# Autodesk Inventor assembly: vertical plate ass
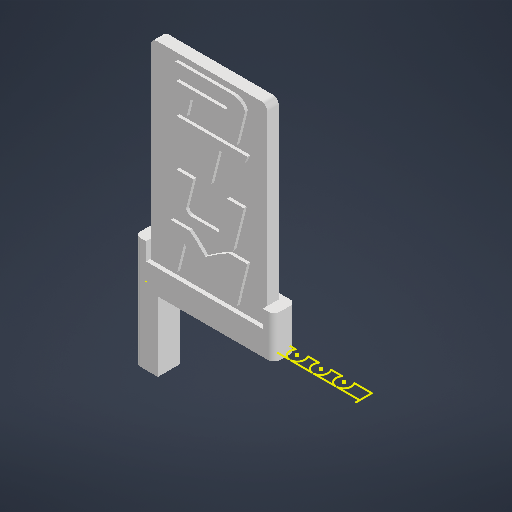
[picture p0: Inventor's stored thumbnail of the model, 512x512]
Saved by Autodesk Inventor 2025.1 (Build 291241000, 241)
## iProperties
Created: 2025-01-21
Part Number: vertical plate ass
Document SubType Name: Assembly
Designer: Juanl
Author: Juanl
## Documents named in this file (3)
- C:\Users\Juanl\Documents\GitHub\ATUM-V5RC-High-Stakes-CAD\Protobot\Hunter Mathis\vertical plate ass.iam
- C:\Users\Juanl\Documents\GitHub\ATUM-V5RC-High-Stakes-CAD\Protobot\Hunter Mathis\plate holder vertical.ipt
- C:\Users\Juanl\Documents\GitHub\ATUM-V5RC-High-Stakes-CAD\Protobot\Hunter Mathis\custom  plate vertical.ipt
## Components (2 placed, 2 different names)
1. plate holder vertical:1 — Mate:1, Mate:2, Mate:3
2. custom  plate vertical:1 — Mate:1, Mate:2, Mate:3
## Relationships (3: Mate 3)
- Mate:1: plate holder vertical:1 ↔ custom  plate vertical:1
- Mate:2: plate holder vertical:1 ↔ custom  plate vertical:1
- Mate:3: plate holder vertical:1 ↔ custom  plate vertical:1
